# Autodesk Inventor assembly: OGAS_01_25_2
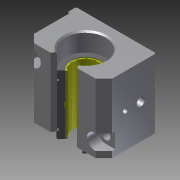
[picture p0: Inventor's stored thumbnail of the model, 180x180]
Saved by Autodesk Inventor 2013 (Build 170138000, 138)
## iProperties
Created: 2013-01-23
Part Number: OGAS_01_25_2
Document SubType Name: Assembly
Designer: Arpan
Author: Arpan
## Documents named in this file (4)
- C:\Users\Arpan\Documents\GitHub\frc2013CAD\Imported Components\OGAS_01_25_2\OGAS_01_25_2.iam
- C:\Users\Arpan\Documents\GitHub\frc2013CAD\Imported Components\OGAS_01_25_2\1.ipt
- C:\Users\Arpan\Documents\GitHub\frc2013CAD\Imported Components\OGAS_01_25_2\2.ipt
- C:\Users\Arpan\Documents\GitHub\frc2013CAD\Imported Components\OGAS_01_25_2\3.ipt
## Components (3 placed, 3 different names)
1. 1:1
2. 2:1 — Mate:1
3. 3:1 — Mate:1
## Relationships (1: Mate 1)
- Mate:1: 2:1 ↔ 3:1
